# Autodesk Inventor assembly: Mesa
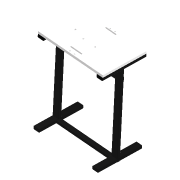
[picture p0: Inventor's stored thumbnail of the model, 180x180]
Saved by Autodesk Inventor 2022 (Build 260153000, 153)
## iProperties
_SolveAssemblyDoc: Frame Generator Solve Assembly
_Version: 25.0.0
Created: 2019-10-25
Part Number: Mesa
Document SubType Name: Assembly
Designer: Usuario
Author: Usuario
## Documents named in this file (5)
- G:\Mi unidad\UTEC\Proyectos\Flor de Lana\Diseño 20191119\Mesa.iam
- G:\Mi unidad\UTEC\Proyectos\Flor de Lana\Diseño 20191119\extructura_mesa.ipt
- G:\Mi unidad\UTEC\Proyectos\Flor de Lana\Diseño 20191119\Mesa\Frame\Frame 1572033469407.iam
- G:\Mi unidad\UTEC\Proyectos\Flor de Lana\Diseño 20191119\Mesa.ipt
- G:\Mi unidad\UTEC\Proyectos\Flor de Lana\Diseño 20191119\Mesa\Frame\Plate Esquinas empalmadas (mm) 1572034518632.ipt
## Components (5 placed, 4 different names)
1. extructura_mesa:1
2. Frame 1572033469407:1 [sub-assembly] — Nivelación:1, Nivelación:2, Coincidencia:1, Rigid:1, Rigid:2
3. Mesa:1 — Nivelación:1, Nivelación:2, Coincidencia:1
4. Esquinas empalmadas (mm) 1 x 50 x 25:1 — Rigid:1
5. Esquinas empalmadas (mm) 1 x 50 x 25:2 — Rigid:2
## Relationships (5: Flush 2, WeldJoint 2, Mate 1)
- Nivelación:1 [Flush]: Frame 1572033469407:1 ↔ Mesa:1
- Nivelación:2 [Flush]: Frame 1572033469407:1 ↔ Mesa:1
- Coincidencia:1 [Mate]: Frame 1572033469407:1 ↔ Mesa:1
- Rigid:1 [WeldJoint]: Frame 1572033469407:1 ↔ Esquinas empalmadas (mm) 1 x 50 x 25:1
- Rigid:2 [WeldJoint]: Frame 1572033469407:1 ↔ Esquinas empalmadas (mm) 1 x 50 x 25:2
